# Autodesk Inventor assembly: Servo Motor MG996R  With Attachments_MIR
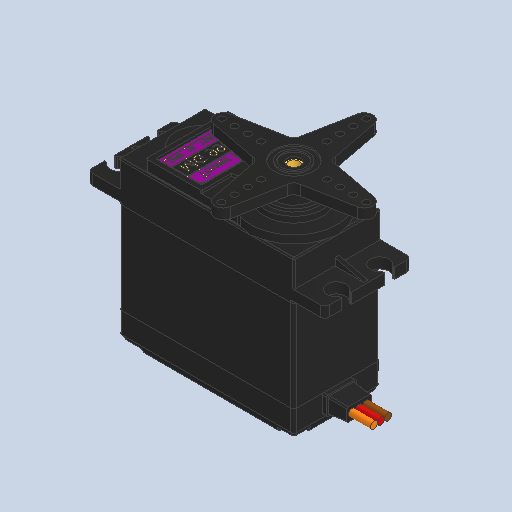
[picture p0: Inventor's stored thumbnail of the model, 512x512]
Saved by Autodesk Inventor 2023 (Build 270158000, 158)
## iProperties
Created: 2023-10-04
Part Number: Servo Motor MG996R  With Attachments_MIR
Document SubType Name: Assembly
Designer: zskus
Sending System: SOLIDWORKS 2016-2016040
MC: AMD64
MC_MODEL: Intel64 Family 6 Model 60 Stepping 3, GenuineIntel
OS: Windows_NT
FRU: Parasolid Version 28.0, build 204, 11- 9-2015
FORMAT: text
GUISE: transmit
KEY: Servo Motor MG996R  With Attachments
FILE: Servo Motor MG996R  With Attachments.x_t
DATE: Tue Oct 27 20:35:35 2020
Author: zskus
## Documents named in this file (14)
- C:\Users\zskus\Desktop\Folders\Personal Projects\Inventor\Project_1_Scooter\Parts\Servo Motor MG996R  With Attachments_MIR.iam
- C:\Users\zskus\Desktop\Folders\Personal Projects\Inventor\Project_1_Scooter\Parts\servoMotorMG996R_MIR.ipt
- C:\Users\zskus\Desktop\Folders\Personal Projects\Inventor\Project_1_Scooter\Parts\servoMotorMG996R_1_MIR.ipt
- C:\Users\zskus\Desktop\Folders\Personal Projects\Inventor\Project_1_Scooter\Parts\servoMotorMG996R_2_MIR.ipt
- C:\Users\zskus\Desktop\Folders\Personal Projects\Inventor\Project_1_Scooter\Parts\servoMotorMG996R_3_MIR.ipt
- C:\Users\zskus\Desktop\Folders\Personal Projects\Inventor\Project_1_Scooter\Parts\servoMotorMG996R_4_MIR.ipt
- C:\Users\zskus\Desktop\Folders\Personal Projects\Inventor\Project_1_Scooter\Parts\servoMotorMG996R_5_MIR.ipt
- C:\Users\zskus\Desktop\Folders\Personal Projects\Inventor\Project_1_Scooter\Parts\servoMotorMG996R_6_MIR.ipt
- C:\Users\zskus\Desktop\Folders\Personal Projects\Inventor\Project_1_Scooter\Parts\servoMotorMG996R_7_MIR.ipt
- C:\Users\zskus\Desktop\Folders\Personal Projects\Inventor\Project_1_Scooter\Parts\attachmentCircular.ipt
- C:\Users\zskus\Desktop\Folders\Personal Projects\Inventor\Project_1_Scooter\Parts\attachmentCircular_1.ipt
- C:\Users\zskus\Desktop\Folders\Personal Projects\Inventor\Project_1_Scooter\Parts\attachmentCross_MIR.ipt
- C:\Users\zskus\Desktop\Folders\Personal Projects\Inventor\Project_1_Scooter\Parts\attachmentStar.ipt
- C:\Users\zskus\Desktop\Folders\Personal Projects\Inventor\Project_1_Scooter\Parts\attachmentStraight.ipt
## Components (13 placed, 13 different names)
1. servoMotorMG996R_MIR:1 — Mate:6, Flush:4, Flush:3, Mate:2, Flush:2, Flush:1
2. servoMotorMG996R_1_MIR:1 — Mate:6, Flush:4, Flush:3
3. servoMotorMG996R_2_MIR:1
4. servoMotorMG996R_3_MIR:1
5. servoMotorMG996R_4_MIR:1
6. servoMotorMG996R_5_MIR:1
7. servoMotorMG996R_6_MIR:1 — Mate:4, Mate:3, Mate:8
8. servoMotorMG996R_7_MIR:1 — Mate:4, Mate:3, Mate:2, Flush:2, Flush:1, Mate:7
9. attachmentCircular:1
10. attachmentCircular_1:1
11. attachmentCross_MIR:1 — Mate:8, Mate:7
12. attachmentStar:1
13. attachmentStraight:1
## Relationships (10: Mate 6, Flush 4)
- Mate:6: servoMotorMG996R_MIR:1 ↔ servoMotorMG996R_1_MIR:1
- Flush:4: servoMotorMG996R_MIR:1 ↔ servoMotorMG996R_1_MIR:1
- Flush:3: servoMotorMG996R_MIR:1 ↔ servoMotorMG996R_1_MIR:1
- Mate:4: servoMotorMG996R_6_MIR:1 ↔ servoMotorMG996R_7_MIR:1
- Mate:3: servoMotorMG996R_6_MIR:1 ↔ servoMotorMG996R_7_MIR:1
- Mate:2: servoMotorMG996R_MIR:1 ↔ servoMotorMG996R_7_MIR:1
- Flush:2: servoMotorMG996R_MIR:1 ↔ servoMotorMG996R_7_MIR:1
- Flush:1: servoMotorMG996R_MIR:1 ↔ servoMotorMG996R_7_MIR:1
- Mate:8: servoMotorMG996R_6_MIR:1 ↔ attachmentCross_MIR:1
- Mate:7: servoMotorMG996R_7_MIR:1 ↔ attachmentCross_MIR:1
